# Autodesk Inventor assembly: KBHandle
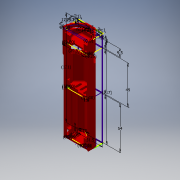
[picture p0: Inventor's stored thumbnail of the model, 180x180]
Saved by Autodesk Inventor 2017 SP1 (Build 210196100, 196)
## iProperties
Created: 2014-08-19
Part Number: KBHandle
Document SubType Name: Assembly
Designer: jkao
Mass: 43.2006 g
Surface Area: 368.135 cm^2
Volume: 40.7553 cm^3
Density: 1.06 g/cm^3
Author: jkao
## Documents named in this file (4)
- H:\Dropbox\projects\inventor\KBHandle\KBHandle.iam
- H:\Dropbox\projects\inventor\KBHandle\DiffuserCoupler.ipt
- H:\Dropbox\projects\inventor\KBHandle\Handle-Bottom.ipt
- H:\Dropbox\projects\inventor\KBHandle\Handle-Top.ipt
## Components (3 placed, 3 different names)
1. DiffuserCoupler:1
2. Handle-Bottom:1 — Flush:1
3. Handle-Top:1 — Flush:1
## Relationships (1: Flush 1)
- Flush:1: Handle-Bottom:1 ↔ Handle-Top:1
